# Autodesk Inventor assembly: UpperArm
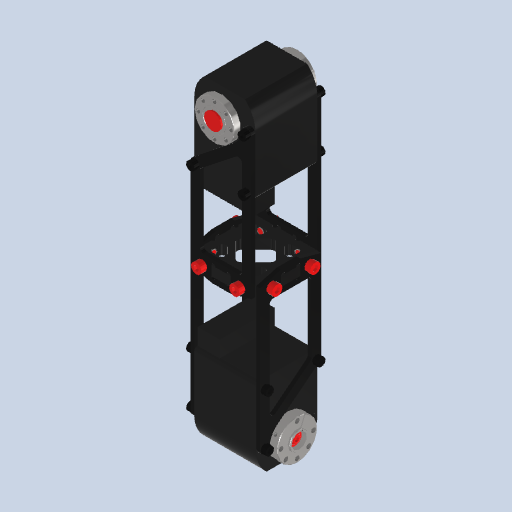
[picture p0: Inventor's stored thumbnail of the model, 512x512]
Saved by Autodesk Inventor 2022 (Build 260153000, 153)
## iProperties
Created: 2021-09-11
Part Number: UpperArm
Document SubType Name: Assembly
Designer: Masato
Mass: 132.402 g
Surface Area: 432.665 cm^2
Volume: 110.152 cm^3
Density: 1.20199 g/cm^3
Author: Masato
## Documents named in this file (8)
- C:\Users\MasatoKubotera\Desktop\SUSTAINA-OP\UpperBody\Arm\UpperArm.iam
- C:\Users\MasatoKubotera\Desktop\SUSTAINA-OP\UpperBody\Arm\UpperArm_side_frame.ipt
- C:\Users\MasatoKubotera\Desktop\SUSTAINA-OP\UpperBody\Arm\UpperArm_diagonal.ipt
- C:\Users\MasatoKubotera\Desktop\SUSTAINA-OP\ReadyMade\Screw\FC-2615EB.ipt
- C:\Users\MasatoKubotera\Desktop\SUSTAINA-OP\ReadyMade\Screw\FC-2620EB.ipt
- C:\Users\MasatoKubotera\Desktop\SUSTAINA-OP\ReadyMade\Screw\UC-0306.ipt
- C:\Users\MasatoKubotera\Desktop\SUSTAINA-OP\ReadyMade\InsertNut\IRU-304S.ipt
- C:\Users\MasatoKubotera\Desktop\SUSTAINA-OP\ReadyMade\KONDO\B3M-SC-1040-A_with_ClampHorn_AND_FreeHorn.iam
## Components (35 placed, 7 different names)
1. UpperArm_side_frame:4 — 挿入:6, 挿入:5, 挿入:15, 挿入:16, 挿入:29, 挿入:30, 挿入:31, 挿入:72, 挿入:73, 挿入:76
2. UpperArm_side_frame:3 — 挿入:8, 挿入:7, 挿入:14, 挿入:13, 挿入:35, 挿入:36, 挿入:37, 挿入:77, 挿入:78, 挿入:79
3. UpperArm_side_frame:2 — 挿入:3, 挿入:4, 挿入:11, 挿入:12, 挿入:38, 挿入:39, 挿入:40, 挿入:81, 挿入:82, 挿入:83
4. UpperArm_side_frame:1 — 挿入:1, 挿入:2, 挿入:32, 挿入:33, 挿入:34, 挿入:74, 挿入:75, 挿入:80, 挿入:84, 挿入:85
5. UpperArm_diagonal:1 — 挿入:1, 挿入:2, 挿入:3, 挿入:4, 挿入:5, 挿入:6, 挿入:7, 挿入:8, メイト:3, フラッシュ:1, フラッシュ:2, 挿入:64, 挿入:65, 挿入:66, 挿入:67, 挿入:68, 挿入:69, 挿入:70, 挿入:71
6. B3M-SC-1040-A_with_ClampHorn_AND_FreeHorn:1 [sub-assembly] — 挿入:72, 挿入:73, 挿入:76, 挿入:77, 挿入:78, 挿入:79
7. B3M-SC-1040-A_with_ClampHorn_AND_FreeHorn:2 [sub-assembly] — 挿入:74, 挿入:75, 挿入:80, 挿入:81, 挿入:82, 挿入:83
8. FC-2620EB:6 — 挿入:40
9. FC-2620EB:5 — 挿入:38
10. FC-2620EB:4 — 挿入:39
11. FC-2620EB:3 — 挿入:37
12. FC-2620EB:2 — 挿入:36
13. FC-2620EB:1 — 挿入:35
14. FC-2615EB:6 — 挿入:34
15. FC-2615EB:5 — 挿入:33
16. FC-2615EB:4 — 挿入:32
17. FC-2615EB:3 — 挿入:31
18. FC-2615EB:2 — 挿入:30
19. FC-2615EB:1 — 挿入:29
20. UC-0306:8 — 挿入:16
21. UC-0306:7 — 挿入:15
22. UC-0306:6 — 挿入:14
23. UC-0306:5 — 挿入:13
24. UC-0306:4 — 挿入:12
25. UC-0306:3 — 挿入:11
26. UC-0306:2 — 挿入:85
27. UC-0306:1 — 挿入:84
28. IRU-304S:8 — 挿入:71
29. IRU-304S:7 — 挿入:70
30. IRU-304S:6 — 挿入:69
31. IRU-304S:5 — 挿入:68
32. IRU-304S:4 — 挿入:67
33. IRU-304S:3 — 挿入:66
34. IRU-304S:2 — 挿入:65
35. IRU-304S:1 — 挿入:64
## Relationships (51: Insert 48, Flush 2, Mate 1)
- 挿入:1 [Insert]: UpperArm_side_frame:1 ↔ UpperArm_diagonal:1
- 挿入:2 [Insert]: UpperArm_side_frame:1 ↔ UpperArm_diagonal:1
- 挿入:3 [Insert]: UpperArm_side_frame:2 ↔ UpperArm_diagonal:1
- 挿入:4 [Insert]: UpperArm_side_frame:2 ↔ UpperArm_diagonal:1
- 挿入:5 [Insert]: UpperArm_side_frame:4 ↔ UpperArm_diagonal:1
- 挿入:6 [Insert]: UpperArm_side_frame:4 ↔ UpperArm_diagonal:1
- 挿入:7 [Insert]: UpperArm_side_frame:3 ↔ UpperArm_diagonal:1
- 挿入:8 [Insert]: UpperArm_side_frame:3 ↔ UpperArm_diagonal:1
- 挿入:11 [Insert]: UpperArm_side_frame:2 ↔ UC-0306:3
- 挿入:12 [Insert]: UpperArm_side_frame:2 ↔ UC-0306:4
- 挿入:13 [Insert]: UpperArm_side_frame:3 ↔ UC-0306:5
- 挿入:14 [Insert]: UpperArm_side_frame:3 ↔ UC-0306:6
- 挿入:15 [Insert]: UpperArm_side_frame:4 ↔ UC-0306:7
- 挿入:16 [Insert]: UpperArm_side_frame:4 ↔ UC-0306:8
- 挿入:29 [Insert]: UpperArm_side_frame:4 ↔ FC-2615EB:1
- 挿入:30 [Insert]: UpperArm_side_frame:4 ↔ FC-2615EB:2
- 挿入:31 [Insert]: UpperArm_side_frame:4 ↔ FC-2615EB:3
- 挿入:32 [Insert]: UpperArm_side_frame:1 ↔ FC-2615EB:4
- 挿入:33 [Insert]: UpperArm_side_frame:1 ↔ FC-2615EB:5
- 挿入:35 [Insert]: UpperArm_side_frame:3 ↔ FC-2620EB:1
- 挿入:34 [Insert]: UpperArm_side_frame:1 ↔ FC-2615EB:6
- 挿入:36 [Insert]: UpperArm_side_frame:3 ↔ FC-2620EB:2
- 挿入:37 [Insert]: UpperArm_side_frame:3 ↔ FC-2620EB:3
- 挿入:38 [Insert]: UpperArm_side_frame:2 ↔ FC-2620EB:5
- 挿入:39 [Insert]: UpperArm_side_frame:2 ↔ FC-2620EB:4
- 挿入:40 [Insert]: UpperArm_side_frame:2 ↔ FC-2620EB:6
- メイト:3 [Mate]: UpperArm_diagonal:1
- フラッシュ:1 [Flush]: UpperArm_diagonal:1
- フラッシュ:2 [Flush]: UpperArm_diagonal:1
- 挿入:64 [Insert]: UpperArm_diagonal:1 ↔ IRU-304S:1
- 挿入:65 [Insert]: UpperArm_diagonal:1 ↔ IRU-304S:2
- 挿入:66 [Insert]: UpperArm_diagonal:1 ↔ IRU-304S:3
- 挿入:67 [Insert]: UpperArm_diagonal:1 ↔ IRU-304S:4
- 挿入:68 [Insert]: UpperArm_diagonal:1 ↔ IRU-304S:5
- 挿入:69 [Insert]: UpperArm_diagonal:1 ↔ IRU-304S:6
- 挿入:70 [Insert]: UpperArm_diagonal:1 ↔ IRU-304S:7
- 挿入:71 [Insert]: UpperArm_diagonal:1 ↔ IRU-304S:8
- 挿入:72 [Insert]: UpperArm_side_frame:4 ↔ B3M-SC-1040-A_with_ClampHorn_AND_FreeHorn:1
- 挿入:73 [Insert]: UpperArm_side_frame:4 ↔ B3M-SC-1040-A_with_ClampHorn_AND_FreeHorn:1
- 挿入:74 [Insert]: UpperArm_side_frame:1 ↔ B3M-SC-1040-A_with_ClampHorn_AND_FreeHorn:2
- 挿入:75 [Insert]: UpperArm_side_frame:1 ↔ B3M-SC-1040-A_with_ClampHorn_AND_FreeHorn:2
- 挿入:76 [Insert]: UpperArm_side_frame:4 ↔ B3M-SC-1040-A_with_ClampHorn_AND_FreeHorn:1
- 挿入:77 [Insert]: UpperArm_side_frame:3 ↔ B3M-SC-1040-A_with_ClampHorn_AND_FreeHorn:1
- 挿入:78 [Insert]: UpperArm_side_frame:3 ↔ B3M-SC-1040-A_with_ClampHorn_AND_FreeHorn:1
- 挿入:79 [Insert]: UpperArm_side_frame:3 ↔ B3M-SC-1040-A_with_ClampHorn_AND_FreeHorn:1
- 挿入:80 [Insert]: UpperArm_side_frame:1 ↔ B3M-SC-1040-A_with_ClampHorn_AND_FreeHorn:2
- 挿入:81 [Insert]: UpperArm_side_frame:2 ↔ B3M-SC-1040-A_with_ClampHorn_AND_FreeHorn:2
- 挿入:82 [Insert]: UpperArm_side_frame:2 ↔ B3M-SC-1040-A_with_ClampHorn_AND_FreeHorn:2
- 挿入:83 [Insert]: UpperArm_side_frame:2 ↔ B3M-SC-1040-A_with_ClampHorn_AND_FreeHorn:2
- 挿入:84 [Insert]: UpperArm_side_frame:1 ↔ UC-0306:1
- 挿入:85 [Insert]: UpperArm_side_frame:1 ↔ UC-0306:2
